# Autodesk Inventor assembly: openmv4_h7
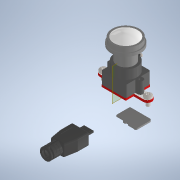
[picture p0: Inventor's stored thumbnail of the model, 180x180]
Saved by Autodesk Inventor 2022 (Build 260153000, 153)
## iProperties
Created: 2019-09-24
Part Number: openmv4_h7
Description: STEP AP214
Document SubType Name: Assembly
Designer: akapu
Sending System: SolidWorks 2016
Preprocessor: SwSTEP 2.0
Title: openmv4_h7.STEP
Revision Number: ANY
## Documents named in this file (8)
- C:\Users\akapu\Documents\maze bot\OpenMV H7\openmv4_h7.iam
- C:\Users\akapu\Documents\maze bot\OpenMV H7\openmv4_ov7725_® ã¬®«ç ­¨î.iam
- C:\Users\akapu\Documents\maze bot\OpenMV H7\pan head cross recess screw_iso_ISO 7045 - M2.5 x 5 - Z - 5N.ipt
- C:\Users\akapu\Documents\maze bot\OpenMV H7\microsd card.ipt
- C:\Users\akapu\Documents\maze bot\OpenMV H7\LENS_Standard_® ã¬®«ç ­¨î.ipt
- C:\Users\akapu\Documents\maze bot\OpenMV H7\LENS_Wide_® ã¬®«ç ­¨î.ipt
- C:\Users\akapu\Documents\maze bot\OpenMV H7\Micro USB connector.ipt
- C:\Users\akapu\Documents\maze bot\OpenMV H7\pan head cross recess screw_iso_ISO 7045 - M1 x 4 - Z - 4S.ipt
## Components (8 placed, 8 different names)
1. openmv4_ov7725_® ã¬®«ç ­¨î_2 [sub-assembly] — Заподлицо:1
2. pan head cross recess screw_iso_ISO 7045 - M2.5 x 5 - Z - 5N_3
3. pan head cross recess screw_iso_ISO 7045 - M2.5 x 5 - Z - 5N_4
4. microsd card_5
5. LENS_Standard_® ã¬®«ç ­¨î_6
6. LENS_Wide_® ã¬®«ç ­¨î_7
7. Micro USB connector_8
8. pan head cross recess screw_iso_ISO 7045 - M1 x 4 - Z - 4S_9
## Relationships (1: Flush 1)
- Заподлицо:1 [Flush] (-8.5 mm): openmv4_ov7725_® ã¬®«ç ­¨î_2
